# Autodesk Inventor assembly: P08_10 Mecanismo 4B
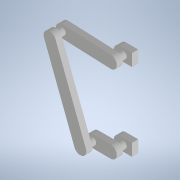
[picture p0: Inventor's stored thumbnail of the model, 180x180]
Saved by Autodesk Inventor 2021 (Build 250183000, 183)
## iProperties
Created: 2021-07-30
Part Number: P08_10 Mecanismo 4B
Document SubType Name: Assembly
Designer: uriel
Author: uriel
## Documents named in this file (6)
- E:\Users\Almanzor\Documents\Escuela\LABORATORIO DISEÑO Y MANUFACTURA ASISTIDA POR COMPUTADORA\Practica 8\BRIDA DE APRIETE\m4b\P08_10 Mecanismo 4B.iam
- E:\Users\Almanzor\Documents\Escuela\LABORATORIO DISEÑO Y MANUFACTURA ASISTIDA POR COMPUTADORA\Practica 8\BRIDA DE APRIETE\m4b\M4B01.ipt
- E:\Users\Almanzor\Documents\Escuela\LABORATORIO DISEÑO Y MANUFACTURA ASISTIDA POR COMPUTADORA\Practica 8\BRIDA DE APRIETE\m4b\M4B02.ipt
- E:\Users\Almanzor\Documents\Escuela\LABORATORIO DISEÑO Y MANUFACTURA ASISTIDA POR COMPUTADORA\Practica 8\BRIDA DE APRIETE\m4b\M4B03.ipt
- E:\Users\Almanzor\Documents\Escuela\LABORATORIO DISEÑO Y MANUFACTURA ASISTIDA POR COMPUTADORA\Practica 8\BRIDA DE APRIETE\m4b\M4B04.ipt
- E:\Users\Almanzor\Documents\Escuela\LABORATORIO DISEÑO Y MANUFACTURA ASISTIDA POR COMPUTADORA\Practica 8\BRIDA DE APRIETE\m4b\M4B05.ipt
## Components (9 placed, 5 different names)
1. M4B01:1 — Insertar:1, Nivelación:1, Nivelación:2, Coincidencia:1, Ángulo:1
2. M4B01:2 — Nivelación:1, Nivelación:2, Coincidencia:1, Insertar:8
3. M4B02:1 — Insertar:6, Insertar:7
4. M4B03:1 — Insertar:2, Insertar:3, Ángulo:1
5. M4B04:1 — Insertar:4, Insertar:5
6. M4B05:1 — Insertar:3, Insertar:4
7. M4B05:2 — Insertar:7, Insertar:8
8. M4B05:4 — Insertar:5, Insertar:6
9. M4B05:5 — Insertar:1, Insertar:2
## Relationships (12: Insert 8, Flush 2, Mate 1, Angle 1)
- Insertar:1: M4B01:1 ↔ M4B05:5
- Insertar:2: M4B03:1 ↔ M4B05:5
- Insertar:3: M4B03:1 ↔ M4B05:1
- Insertar:4: M4B04:1 ↔ M4B05:1
- Insertar:5: M4B04:1 ↔ M4B05:4
- Insertar:6: M4B02:1 ↔ M4B05:4
- Nivelación:1 [Flush]: M4B01:1 ↔ M4B01:2
- Nivelación:2 [Flush]: M4B01:1 ↔ M4B01:2
- Coincidencia:1 [Mate]: M4B01:1 ↔ M4B01:2
- Insertar:7: M4B02:1 ↔ M4B05:2
- Insertar:8: M4B01:2 ↔ M4B05:2
- Ángulo:1 [Angle] (0 deg): M4B01:1 ↔ M4B03:1
